# Autodesk Inventor assembly: FullArm
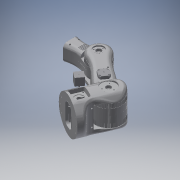
[picture p0: Inventor's stored thumbnail of the model, 180x180]
Saved by Autodesk Inventor 2019 (Build 230136000, 136)
## iProperties
Created: 2020-03-22
Part Number: FullArm
Document SubType Name: Assembly
Designer: james
Author: james
## Documents named in this file (4)
- F:\JimsRobot\FIRSTRobots\Design\RBX1-REMIX\FullArm.iam
- F:\JimsRobot\FIRSTRobots\Design\RBX1-REMIX\forearm\forearm.iam
- F:\JimsRobot\FIRSTRobots\Design\RBX1-REMIX\arm\arm.iam
- F:\JimsRobot\FIRSTRobots\Design\RBX1-REMIX\shoulder\shoulder.iam
## Components (3 placed, 3 different names)
1. forearm:1 [sub-assembly] — Mate:1, Mate:2
2. arm:1 [sub-assembly] — Mate:1, Mate:2, Mate:3, Mate:4
3. shoulder:1 [sub-assembly] — Mate:3, Mate:4
## Relationships (4: Mate 4)
- Mate:1: forearm:1 ↔ arm:1
- Mate:2: forearm:1 ↔ arm:1
- Mate:3: arm:1 ↔ shoulder:1
- Mate:4: arm:1 ↔ shoulder:1
